# Autodesk Inventor assembly: Base Cover Assembly
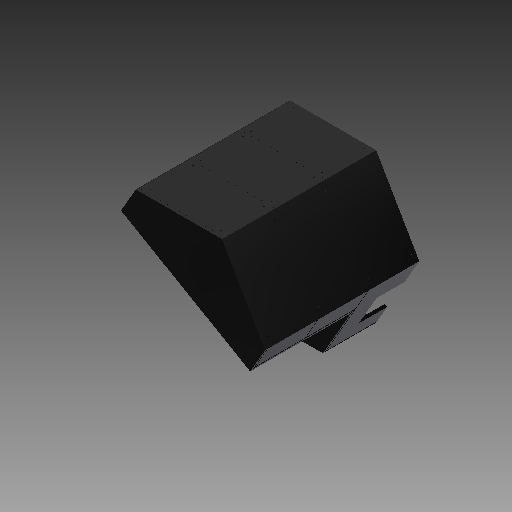
[picture p0: Inventor's stored thumbnail of the model, 512x512]
Saved by Autodesk Inventor 2017 (Build 210142000, 142)
## iProperties
Created: 2018-10-18
Part Number: Base Cover Assembly
Document SubType Name: Assembly
Designer: Dell
Author: Dell
## Documents named in this file (9)
- C:\Users\Dell\Documents\GitHub\tr2\Base\Base Cover Assembly.iam
- C:\Users\Dell\Documents\GitHub\tr2\Base\BA03.ipt
- C:\Users\Dell\Documents\GitHub\tr2\Base\BA04.ipt
- C:\Users\Dell\Documents\GitHub\tr2\BA01.ipt
- C:\Users\Dell\Documents\GitHub\tr2\Base\BA05.ipt
- C:\Users\Dell\Documents\GitHub\tr2\Base\BA09.ipt
- C:\Users\Dell\Documents\GitHub\tr2\Base\BA10.ipt
- C:\Users\Dell\Documents\GitHub\tr2\Base\BA12.ipt
- C:\Users\Dell\Documents\GitHub\tr2\Base\BA13.ipt
## Components (21 placed, 8 different names)
1. BA03:1
2. BA03:2
3. BA03:3
4. BA03:4
5. BA04:1
6. BA01:1
7. BA05:1
8. BA03:5
9. BA03:6
10. BA03:7
11. BA03:8
12. BA09:1
13. BA09:2
14. BA09:3
15. BA09:4
16. BA10:1
17. BA12:1
18. BA12:2
19. BA12:3
20. BA12:4
21. BA13:1
## Relationships (22: Mate 14, Flush 8)
- [Mate]: BA03:3 ↔ BA03:4
- [Mate]: BA03:2 ↔ BA03:5
- [Mate]: BA03:5 ↔ BA03:6
- [Mate]: BA03:7 ↔ BA03:8
- [Mate]: BA03:1 ↔ BA03:7
- [Mate]: BA04:1 ↔ BA09:1
- [Mate]: BA09:1 ↔ BA09:2
- [Mate]: BA09:3 ↔ BA09:4
- [Mate]: BA09:3 ↔ BA09:4
- [Mate]: BA05:1 ↔ BA09:4
- [Mate]: BA04:1 ↔ BA12:1
- [Flush]: BA09:2 ↔ BA12:1
- [Mate]: BA05:1 ↔ BA12:2
- [Flush]: BA09:4 ↔ BA12:2
- [Flush]: BA09:3 ↔ BA12:3
- [Mate]: BA12:2 ↔ BA12:3
- [Flush]: BA09:2 ↔ BA12:4
- [Mate]: BA12:1 ↔ BA12:4
- [Flush]: BA03:6 ↔ BA13:1
- [Flush]: BA03:8 ↔ BA13:1
- [Flush]: BA03:4 ↔ BA10:1
- [Flush]: BA03:3 ↔ BA10:1
## Named parameters: d150_d147 = 0 mm, d131_d130 = 0 mm
